# Autodesk Inventor assembly: W686ZZ
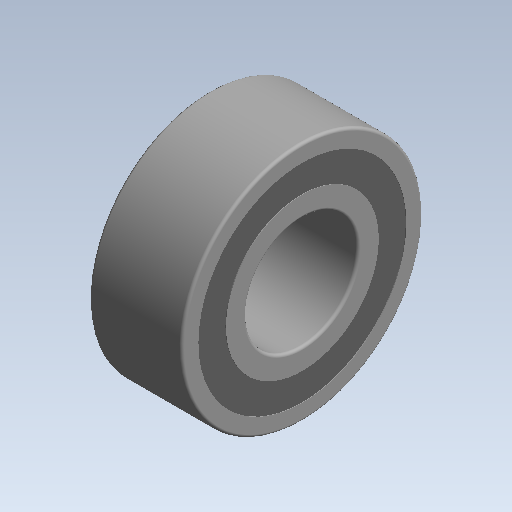
[picture p0: Inventor's stored thumbnail of the model, 512x512]
Saved by Autodesk Inventor 2021.3 (Build 253353010, 353A)
## iProperties
Part Number: W686ZZ
Catalog Web Link: www.cadenas.de
Description: With double shield ZZ-
Vendor: NTN
Document SubType Name: Assembly
Designer: partserver
Manufacturer: NTN
Mass: 0.34909 g
Surface Area: 10.3811 cm^2
Volume: 0.34909 cm^3
Density: 1 g/cm^3
Category: PARTsolutions
Company: NTN
PSOL_IDENT_0: {$CADENAS_DATA\23d-libs\ntn\ball_roller_bearings\miniature_extra_small_bb\metric_system_sizes\mss_zz
PSOL_IDENT_1: _asmtab.prj},184 {VTYP=3D},{STYP=ASSTAB},{NB=W686ZZ},{LINA=W686ZZ},{NN=With double shield ZZ},{DATE=
PSOL_IDENT_2: 23.10.2020 01:13:34},{GEOMDATE=10.03.2020 01:14:46},{VERSION=},{LINEID=12860},{WBVAR=},{WBNUMERIC=}
PSOL_IDENT_3: {NB=W686ZZ},{LINA=W686ZZ},{KT=DUMMY},{IDNR=},{SD=6.0},{D=13},{B=3.5},{B1=5.0},{D1=15.0},{D2=15.2},{
PSOL_IDENT_4: C1=1.0},{C2=1.1},{R=0.15},{ORDER=W686ZZ},{CR=1200},{COR=440},{CU=17.5},{CRF=110},{CORF=45},{LSG=39 0
PSOL_IDENT_5: 00},{LSO=46 000},{MASS=1.90},{ORDER1=686},{WSS=W686ZZ},{WDS=ZZ},{UTWF=FL686},{FORSS=FLW686Z},{FORDS=
PSOL_IDENT_6: ZZ},{DA1=7},{DA2=7,2},{DA=11,8},{RAS=0,15},{MASS1=2.20},{VERS=3},{X=3.5},{N=8},{O=29.83},{RB=1.036},
PSOL_IDENT_7: {PPATH=mss_asmtpl.prj}
NB: W686ZZ
NN: With double shield ZZ
NBSYN: $ORDER.
LINA: W686ZZ
CATALOG: NTN Corporation
SD: 6
D: 13
B1: 5
R: 0.15
ORDER: W686ZZ
CR: 1200
COR: 440
CU: 17.5
LSG: 39 000
LSO: 46 000
MASS: 1.9
SUPPLIER: NTN
ARTICLENO: W686ZZ
BOMINFO: W686ZZ
CREATOR: CADENAS GmbH
Title: W686ZZ
Author: Cadenas PARTsolutions
## Documents named in this file (5)
- C:\Users\YusukeKunita\Documents\GrabCAD\NHK2021\BasicParts\よく使う部品（萩原）\Bearing\NTN686\W686ZZ.iam
- C:\Users\YusukeKunita\Documents\GrabCAD\NHK2021\BasicParts\よく使う部品（萩原）\Bearing\NTN686\W686ZZ Inner ring.ipt
- C:\Users\YusukeKunita\Documents\GrabCAD\NHK2021\BasicParts\よく使う部品（萩原）\Bearing\NTN686\W686ZZ Outer ring.ipt
- C:\Users\YusukeKunita\Documents\GrabCAD\NHK2021\BasicParts\よく使う部品（萩原）\Bearing\NTN686\W686ZZ Shield.ipt
- C:\Users\YusukeKunita\Documents\GrabCAD\NHK2021\BasicParts\よく使う部品（萩原）\Bearing\NTN686\W686ZZ Ball.ipt
## Components (12 placed, 4 different names)
1. W686ZZ Inner ring:1 — mss_ir_Z@1 <-> mss_or_Z@2
2. W686ZZ Outer ring:1 — mss_ir_Z@1 <-> mss_or_Z@2, mss_or_XY@2 <-> mss_s_XY@3, mss_or_Z@2 <-> mss_s_Z@3, mss_or_YZ@2 <-> mss_s_YZ@3, mss_or11_XY@2 <-> mss_s_XY@4, mss_or11_Z@2 <-> mss_s_Z@4, mss_or11_YZ@2 <-> mss_s_YZ@4, mss_or21_1_XY@2 <-> mss_ball_XY@5, mss_or21_1_Z@2 <-> mss_ball_Z@5, mss_or21_1_YZ@2 <-> mss_ball_YZ@5, mss_or21_2_XY@2 <-> mss_ball_XY@6, mss_or21_2_Z@2 <-> mss_ball_Z@6, mss_or21_2_YZ@2 <-> mss_ball_YZ@6, mss_or21_3_XY@2 <-> mss_ball_XY@7, mss_or21_3_Z@2 <-> mss_ball_Z@7, mss_or21_3_YZ@2 <-> mss_ball_YZ@7, mss_or21_4_XY@2 <-> mss_ball_XY@8, mss_or21_4_Z@2 <-> mss_ball_Z@8, mss_or21_4_YZ@2 <-> mss_ball_YZ@8, mss_or21_5_XY@2 <-> mss_ball_XY@9, mss_or21_5_Z@2 <-> mss_ball_Z@9, mss_or21_5_YZ@2 <-> mss_ball_YZ@9, mss_or21_6_XY@2 <-> mss_ball_XY@10, mss_or21_6_Z@2 <-> mss_ball_Z@10, mss_or21_6_YZ@2 <-> mss_ball_YZ@10, mss_or21_7_XY@2 <-> mss_ball_XY@11, mss_or21_7_Z@2 <-> mss_ball_Z@11, mss_or21_7_YZ@2 <-> mss_ball_YZ@11, mss_or21_8_XY@2 <-> mss_ball_XY@12, mss_or21_8_Z@2 <-> mss_ball_Z@12, mss_or21_8_YZ@2 <-> mss_ball_YZ@12
3. W686ZZ Shield:1 — mss_or_XY@2 <-> mss_s_XY@3, mss_or_Z@2 <-> mss_s_Z@3, mss_or_YZ@2 <-> mss_s_YZ@3
4. W686ZZ Shield:2 — mss_or11_XY@2 <-> mss_s_XY@4, mss_or11_Z@2 <-> mss_s_Z@4, mss_or11_YZ@2 <-> mss_s_YZ@4
5. W686ZZ Ball:1 — mss_or21_1_XY@2 <-> mss_ball_XY@5, mss_or21_1_Z@2 <-> mss_ball_Z@5, mss_or21_1_YZ@2 <-> mss_ball_YZ@5
6. W686ZZ Ball:2 — mss_or21_2_XY@2 <-> mss_ball_XY@6, mss_or21_2_Z@2 <-> mss_ball_Z@6, mss_or21_2_YZ@2 <-> mss_ball_YZ@6
7. W686ZZ Ball:3 — mss_or21_3_XY@2 <-> mss_ball_XY@7, mss_or21_3_Z@2 <-> mss_ball_Z@7, mss_or21_3_YZ@2 <-> mss_ball_YZ@7
8. W686ZZ Ball:4 — mss_or21_4_XY@2 <-> mss_ball_XY@8, mss_or21_4_Z@2 <-> mss_ball_Z@8, mss_or21_4_YZ@2 <-> mss_ball_YZ@8
9. W686ZZ Ball:5 — mss_or21_5_XY@2 <-> mss_ball_XY@9, mss_or21_5_Z@2 <-> mss_ball_Z@9, mss_or21_5_YZ@2 <-> mss_ball_YZ@9
10. W686ZZ Ball:6 — mss_or21_6_XY@2 <-> mss_ball_XY@10, mss_or21_6_Z@2 <-> mss_ball_Z@10, mss_or21_6_YZ@2 <-> mss_ball_YZ@10
11. W686ZZ Ball:7 — mss_or21_7_XY@2 <-> mss_ball_XY@11, mss_or21_7_Z@2 <-> mss_ball_Z@11, mss_or21_7_YZ@2 <-> mss_ball_YZ@11
12. W686ZZ Ball:8 — mss_or21_8_XY@2 <-> mss_ball_XY@12, mss_or21_8_Z@2 <-> mss_ball_Z@12, mss_or21_8_YZ@2 <-> mss_ball_YZ@12
## Relationships (31: Mate 20, Angle 10, Flush 1)
- mss_ir_Z@1 <-> mss_or_Z@2 [Mate]: W686ZZ Inner ring:1 ↔ W686ZZ Outer ring:1
- mss_or_XY@2 <-> mss_s_XY@3 [Mate]: W686ZZ Outer ring:1 ↔ W686ZZ Shield:1
- mss_or_Z@2 <-> mss_s_Z@3 [Mate]: W686ZZ Outer ring:1 ↔ W686ZZ Shield:1
- mss_or_YZ@2 <-> mss_s_YZ@3 [Angle] (0 deg): W686ZZ Outer ring:1 ↔ W686ZZ Shield:1
- mss_or11_XY@2 <-> mss_s_XY@4 [Flush]: W686ZZ Outer ring:1 ↔ W686ZZ Shield:2
- mss_or11_Z@2 <-> mss_s_Z@4 [Mate]: W686ZZ Outer ring:1 ↔ W686ZZ Shield:2
- mss_or11_YZ@2 <-> mss_s_YZ@4 [Angle] (0 deg): W686ZZ Outer ring:1 ↔ W686ZZ Shield:2
- mss_or21_1_XY@2 <-> mss_ball_XY@5 [Mate]: W686ZZ Outer ring:1 ↔ W686ZZ Ball:1
- mss_or21_1_Z@2 <-> mss_ball_Z@5 [Mate]: W686ZZ Outer ring:1 ↔ W686ZZ Ball:1
- mss_or21_1_YZ@2 <-> mss_ball_YZ@5 [Angle] (0 deg): W686ZZ Outer ring:1 ↔ W686ZZ Ball:1
- mss_or21_2_XY@2 <-> mss_ball_XY@6 [Mate]: W686ZZ Outer ring:1 ↔ W686ZZ Ball:2
- mss_or21_2_Z@2 <-> mss_ball_Z@6 [Mate]: W686ZZ Outer ring:1 ↔ W686ZZ Ball:2
- mss_or21_2_YZ@2 <-> mss_ball_YZ@6 [Angle] (0 deg): W686ZZ Outer ring:1 ↔ W686ZZ Ball:2
- mss_or21_3_XY@2 <-> mss_ball_XY@7 [Mate]: W686ZZ Outer ring:1 ↔ W686ZZ Ball:3
- mss_or21_3_Z@2 <-> mss_ball_Z@7 [Mate]: W686ZZ Outer ring:1 ↔ W686ZZ Ball:3
- mss_or21_3_YZ@2 <-> mss_ball_YZ@7 [Angle] (0 deg): W686ZZ Outer ring:1 ↔ W686ZZ Ball:3
- mss_or21_4_XY@2 <-> mss_ball_XY@8 [Mate]: W686ZZ Outer ring:1 ↔ W686ZZ Ball:4
- mss_or21_4_Z@2 <-> mss_ball_Z@8 [Mate]: W686ZZ Outer ring:1 ↔ W686ZZ Ball:4
- mss_or21_4_YZ@2 <-> mss_ball_YZ@8 [Angle] (0 deg): W686ZZ Outer ring:1 ↔ W686ZZ Ball:4
- mss_or21_5_XY@2 <-> mss_ball_XY@9 [Mate]: W686ZZ Outer ring:1 ↔ W686ZZ Ball:5
- mss_or21_5_Z@2 <-> mss_ball_Z@9 [Mate]: W686ZZ Outer ring:1 ↔ W686ZZ Ball:5
- mss_or21_5_YZ@2 <-> mss_ball_YZ@9 [Angle] (0 deg): W686ZZ Outer ring:1 ↔ W686ZZ Ball:5
- mss_or21_6_XY@2 <-> mss_ball_XY@10 [Mate]: W686ZZ Outer ring:1 ↔ W686ZZ Ball:6
- mss_or21_6_Z@2 <-> mss_ball_Z@10 [Mate]: W686ZZ Outer ring:1 ↔ W686ZZ Ball:6
- mss_or21_6_YZ@2 <-> mss_ball_YZ@10 [Angle] (0 deg): W686ZZ Outer ring:1 ↔ W686ZZ Ball:6
- mss_or21_7_XY@2 <-> mss_ball_XY@11 [Mate]: W686ZZ Outer ring:1 ↔ W686ZZ Ball:7
- mss_or21_7_Z@2 <-> mss_ball_Z@11 [Mate]: W686ZZ Outer ring:1 ↔ W686ZZ Ball:7
- mss_or21_7_YZ@2 <-> mss_ball_YZ@11 [Angle] (0 deg): W686ZZ Outer ring:1 ↔ W686ZZ Ball:7
- mss_or21_8_XY@2 <-> mss_ball_XY@12 [Mate]: W686ZZ Outer ring:1 ↔ W686ZZ Ball:8
- mss_or21_8_Z@2 <-> mss_ball_Z@12 [Mate]: W686ZZ Outer ring:1 ↔ W686ZZ Ball:8
- mss_or21_8_YZ@2 <-> mss_ball_YZ@12 [Angle] (0 deg): W686ZZ Outer ring:1 ↔ W686ZZ Ball:8
